# Autodesk Inventor assembly: Rostizador
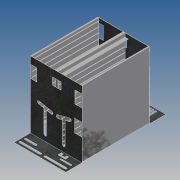
[picture p0: Inventor's stored thumbnail of the model, 180x180]
Saved by Autodesk Inventor 2016 (Build 200138000, 138)
## iProperties
Created: 2016-05-26
Part Number: Rostizador
Document SubType Name: Assembly
Designer: Familia
Author: Familia
## Documents named in this file (4)
- C:\Users\Familia\Desktop\Tostadora\Ensambles\Rostizador.iam
- C:\Users\Familia\Desktop\Tostadora\Partes\Platina forntal interna.ipt
- C:\Users\Familia\Desktop\Tostadora\Partes\Platina lateral interna 2.ipt
- C:\Users\Familia\Desktop\Tostadora\Partes\Platina lateral interna 1.ipt
## Components (6 placed, 3 different names)
1. Platina forntal interna:1 — Flush:1, Mate:1, Flush:2, Mate:2, Flush:3, Mate:3, Mate:4, Mate:5, Mate:6, Flush:4, Flush:7, Flush:9
2. Platina forntal interna:2 — Mate:2, Flush:3, Mate:3, Flush:8
3. Platina lateral interna 2:1 — Mate:4, Mate:6, Mate:7
4. Platina lateral interna 1:1 — Mate:5, Flush:4, Flush:5, Flush:6, Flush:10
5. Platina forntal interna:3 — Flush:6, Flush:7, Flush:9
6. Platina forntal interna:4 — Flush:8, Mate:11, Flush:10
## Relationships (18: Flush 10, Mate 8)
- Flush:1: Platina forntal interna:1
- Mate:1: Platina forntal interna:1
- Flush:2: Platina forntal interna:1
- Mate:2: Platina forntal interna:1 ↔ Platina forntal interna:2
- Flush:3: Platina forntal interna:1 ↔ Platina forntal interna:2
- Mate:3: Platina forntal interna:1 ↔ Platina forntal interna:2
- Mate:4: Platina forntal interna:1 ↔ Platina lateral interna 2:1
- Mate:5: Platina forntal interna:1 ↔ Platina lateral interna 1:1
- Mate:6: Platina forntal interna:1 ↔ Platina lateral interna 2:1
- Flush:4: Platina forntal interna:1 ↔ Platina lateral interna 1:1
- Mate:7: Platina lateral interna 2:1
- Flush:5: Platina lateral interna 1:1
- Flush:6: Platina lateral interna 1:1 ↔ Platina forntal interna:3
- Flush:7: Platina forntal interna:1 ↔ Platina forntal interna:3
- Flush:8: Platina forntal interna:2 ↔ Platina forntal interna:4
- Flush:9: Platina forntal interna:1 ↔ Platina forntal interna:3
- Mate:11: Platina forntal interna:4
- Flush:10: Platina lateral interna 1:1 ↔ Platina forntal interna:4
